# Autodesk Inventor assembly: szafka
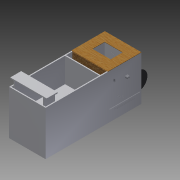
[picture p0: Inventor's stored thumbnail of the model, 180x180]
Saved by Autodesk Inventor 2013 (Build 170138000, 138)
## iProperties
Created: 2014-04-26
Part Number: szafka
Document SubType Name: Assembly
Designer: Masta
Author: Masta
## Documents named in this file (17)
- E:\3d_printer\szafka\szafka.iam
- E:\3d_printer\szafka\bok.ipt
- E:\3d_printer\szafka\tyl.ipt
- E:\3d_printer\szafka\podstawa.ipt
- E:\3d_printer\szafka\polka.ipt
- E:\3d_printer\szafka\rolka_filamentu.ipt
- E:\3d_printer\szafka\gora.ipt
- E:\3d_printer\szafka\listwa_do_szpulek.ipt
- E:\3d_printer\szafka\srodek.ipt
- E:\3d_printer\szafka\polka2.ipt
- E:\3d_printer\szafka\polka-tyl.ipt
- E:\3d_printer\szafka\bok2.ipt
- E:\3d_printer\prusa_i3plus.iam
- E:\3d_printer\szafka\drzwiczki-bok.ipt
- E:\3d_printer\szafka\drzwiczki-przod.ipt
- E:\3d_printer\szafka\listwa1.ipt
- E:\3d_printer\szafka\szuflada150x400mm.iam
## Components (34 placed, 16 different names)
1. bok:1 — Flush:5, Mate:5, Flush:7, Mate:10, Flush:9, Mate:16, Mate:17, Mate:21, Mate:23, Mate:26, Mate:35
2. tyl:1 — Mate:1, Flush:6, Mate:5, Flush:7, Mate:9, Flush:10, Mate:30, Tangent:4, Mate:33, Mate:34, Angle:1
3. podstawa:1 — Flush:5, Flush:6, Mate:16, Tangent:1, Mate:18, Flush:11, Mate:20, Flush:12, Mate:28, Flush:13, Zestawiający:39
4. polka:1 — Mate:9, Mate:10, Mate:15, Mate:24, Mate:29, Mate:37, Mate:38, Flush:18
5. gora:1 — Flush:9, Flush:10, Mate:15, Tangent:3, Flush:16, Mate:31, Mate:33, Mate:36, Angle:2
6. srodek:1 — Mate:20, Mate:21, Flush:12, Mate:22, Mate:25, Mate:32
7. polka2:1 — Mate:22, Mate:23, Mate:24
8. bok2:1 — Mate:28, Flush:13, Flush:15, Mate:31, Mate:32, Flush:17, Równoległy:19
9. prusa_i3plus:1 [sub-assembly] — Mate:29, Mate:30, Flush:15
10. rolka_filamentu:18 — Tangent:3, Tangent:4, Flush:16
11. drzwiczki-bok:1 — Mate:34, Mate:35, Angle:1
12. drzwiczki-przod:1 — Mate:36, Angle:2, Flush:17
13. listwa1:1 — Mate:37, Mate:38, Flush:18
14. szuflada150x400mm:1 [sub-assembly] — Równoległy:19, Zestawiający:39
15. rolka_filamentu:3 — Tangent:1, Tangent:2
16. rolka_filamentu:4 — Mate:17
17. rolka_filamentu:5
18. rolka_filamentu:6
19. rolka_filamentu:7
20. rolka_filamentu:8
21. rolka_filamentu:9
22. rolka_filamentu:10
23. rolka_filamentu:11
24. rolka_filamentu:12
25. rolka_filamentu:13
26. rolka_filamentu:14
27. rolka_filamentu:15
28. rolka_filamentu:16
29. rolka_filamentu:17
30. listwa_do_szpulek:1 — Mate:18, Flush:11, Tangent:2
31. listwa_do_szpulek:2 — Mate:27
32. listwa_do_szpulek:3
33. polka-tyl:1 — Mate:25, Mate:26, Mate:27
34. polka-tyl:2
## Component patterns: (15 elements, first: rolka_filamentu:3), (3 elements, first: listwa_do_szpulek:1), (2 elements, first: polka-tyl:1)
## Relationships (47: Mate 28, Flush 13, Tangent 4, Angle 2)
- Mate:1: tyl:1
- Flush:5: bok:1 ↔ podstawa:1
- Flush:6: tyl:1 ↔ podstawa:1
- Mate:5: bok:1 ↔ tyl:1
- Flush:7: bok:1 ↔ tyl:1
- Mate:9: tyl:1 ↔ polka:1
- Mate:10: bok:1 ↔ polka:1
- Flush:9: bok:1 ↔ gora:1
- Flush:10: tyl:1 ↔ gora:1
- Mate:15 (520 mm): polka:1 ↔ gora:1
- Mate:16: bok:1 ↔ podstawa:1
- Tangent:1: podstawa:1 ↔ rolka_filamentu:3
- Mate:17 (20 mm): bok:1 ↔ rolka_filamentu:4
- Mate:18: podstawa:1 ↔ listwa_do_szpulek:1
- Flush:11 (40 mm): podstawa:1 ↔ listwa_do_szpulek:1
- Tangent:2: rolka_filamentu:3 ↔ listwa_do_szpulek:1
- Mate:20: podstawa:1 ↔ srodek:1
- Mate:21: bok:1 ↔ srodek:1
- Flush:12 (310 mm): podstawa:1 ↔ srodek:1
- Mate:22: srodek:1 ↔ polka2:1
- Mate:23: bok:1 ↔ polka2:1
- Mate:24 (100 mm): polka:1 ↔ polka2:1
- Mate:25: srodek:1 ↔ polka-tyl:1
- Mate:26: bok:1 ↔ polka-tyl:1
- Mate:27: listwa_do_szpulek:2 ↔ polka-tyl:1
- Mate:28: podstawa:1 ↔ bok2:1
- Flush:13: podstawa:1 ↔ bok2:1
- Mate:29: polka:1 ↔ prusa_i3plus:1
- Mate:30 (300 mm): tyl:1 ↔ prusa_i3plus:1
- Flush:15 (100 mm): bok2:1 ↔ prusa_i3plus:1
- Tangent:3: gora:1 ↔ rolka_filamentu:18
- Tangent:4: tyl:1 ↔ rolka_filamentu:18
- Flush:16 (200 mm): gora:1 ↔ rolka_filamentu:18
- Mate:31: gora:1 ↔ bok2:1
- Mate:32: srodek:1 ↔ bok2:1
- Mate:33: tyl:1 ↔ gora:1
- Mate:34: tyl:1 ↔ drzwiczki-bok:1
- Mate:35 (1 mm): bok:1 ↔ drzwiczki-bok:1
- Angle:1 (270 deg): tyl:1 ↔ drzwiczki-bok:1
- Mate:36: gora:1 ↔ drzwiczki-przod:1
- Angle:2 (90 deg): gora:1 ↔ drzwiczki-przod:1
- Flush:17: bok2:1 ↔ drzwiczki-przod:1
- Mate:37: polka:1 ↔ listwa1:1
- Mate:38: polka:1 ↔ listwa1:1
- Flush:18: polka:1 ↔ listwa1:1
- Równoległy:19 [Flush]: bok2:1 ↔ szuflada150x400mm:1
- Zestawiający:39 [Mate]: podstawa:1 ↔ szuflada150x400mm:1
